# Autodesk Inventor assembly: Manish
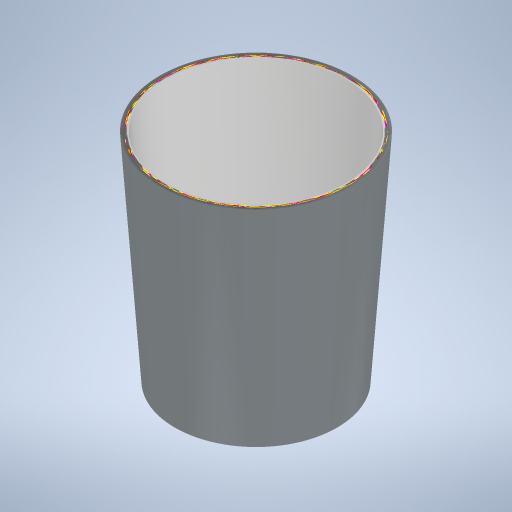
[picture p0: Inventor's stored thumbnail of the model, 512x512]
Saved by Autodesk Inventor 2024 (Build 280153000, 153)
## iProperties
Created: 2024-05-08
Part Number: Manish
Document SubType Name: Assembly
Designer: VIJAY
Author: VIJAY
## Documents named in this file (8)
- C:\Users\VIJAY\OneDrive\Dokumen\Manish.iam
- C:\Users\VIJAY\OneDrive\Dokumen\A.ipt
- C:\Users\VIJAY\OneDrive\Dokumen\B.ipt
- C:\Users\VIJAY\OneDrive\Dokumen\C.ipt
- C:\Users\VIJAY\OneDrive\Dokumen\D.ipt
- C:\Users\VIJAY\OneDrive\Dokumen\E.ipt
- C:\Users\VIJAY\OneDrive\Dokumen\F.ipt
- C:\Users\VIJAY\OneDrive\Dokumen\G.ipt
## Components (7 placed, 7 different names)
1. A:1 — Insert:1, Insert:2, Insert:3, Insert:4, Insert:5, Insert:6
2. B:1 — Insert:1
3. C:1 — Insert:2
4. D:1 — Insert:3
5. E:1 — Insert:4
6. F:1 — Insert:5
7. G:1 — Insert:6
## Relationships (6: Insert 6)
- Insert:1: A:1 ↔ B:1
- Insert:2: A:1 ↔ C:1
- Insert:3: A:1 ↔ D:1
- Insert:4: A:1 ↔ E:1
- Insert:5: A:1 ↔ F:1
- Insert:6: A:1 ↔ G:1
